# Autodesk Inventor assembly: DeckelParabol
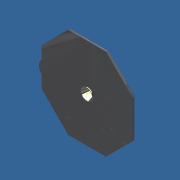
[picture p0: Inventor's stored thumbnail of the model, 180x180]
Saved by Autodesk Inventor 2018.2 (Build 222227000, 227)
## iProperties
Company: Fraunhofer ILT
Created: 2018-10-30
Part Number: DeckelParabol
Material: geeigneten Werkstoff auswählen !
Document SubType Name: Assembly
Designer: N.Grubert
Title: =Description
Author: N.Grubert
## Documents named in this file (3)
- C:\Users\GRUBERT\Documents\COSIMA-Laserstar\CAD\DeckelParabol.iam
- C:\Users\GRUBERT\Documents\COSIMA-Laserstar\CAD\Oktagon_Deckel.ipt
- C:\Users\GRUBERT\Documents\COSIMA-Laserstar\CAD\Parabol.ipt
## Components (2 placed, 2 different names)
1. Oktagon_Deckel:1 — Passend:2
2. Parabol:1 — Passend:1, Passend:2
## Relationships (2: Mate 2)
- Passend:1 [Mate]: Parabol:1
- Passend:2 [Mate]: Oktagon_Deckel:1 ↔ Parabol:1
